# Autodesk Inventor assembly: Airplane_vertical
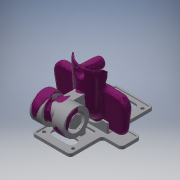
[picture p0: Inventor's stored thumbnail of the model, 180x180]
Saved by Autodesk Inventor 2017 (Build 210142000, 142)
## iProperties
Created: 2017-08-22
Part Number: Airplane_vertical
Document SubType Name: Assembly
Designer: MineV
Author: MineV
## Documents named in this file (3)
- C:\Users\minea\Documents\Vault\vault\Airplane_vertical.iam
- C:\Users\minea\Documents\Vault\vault\Imported Components\rear_mesh\rear_mesh.ipt
- C:\Users\minea\Documents\Vault\vault\Airplane_vertical_holder.ipt
## Components (2 placed, 2 different names)
1. rear_mesh:1 — Mate:2
2. Airplane_vertical_holder:1 — Mate:1
## Relationships (2: Mate 2)
- Mate:1: Airplane_vertical_holder:1
- Mate:2 (44 mm): rear_mesh:1
